# Autodesk Inventor assembly: Chassis_Assembly
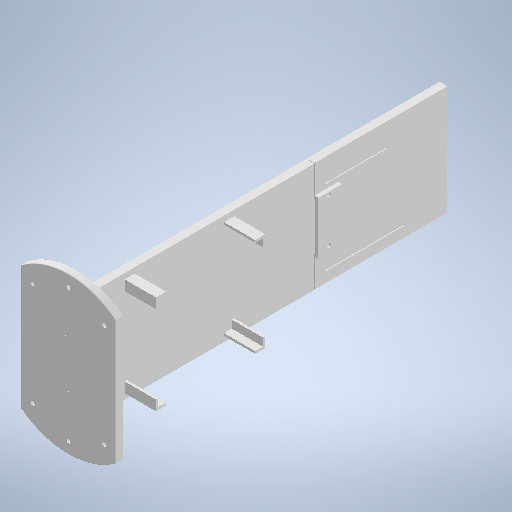
[picture p0: Inventor's stored thumbnail of the model, 512x512]
Saved by Autodesk Inventor 2025 (Build 290162000, 162)
## iProperties
Created: 2024-06-27
Part Number: Chassis_Assembly
Document SubType Name: Assembly
Designer: sml6042
Author: sml6042
## Documents named in this file (4)
- C:\Users\sml6042\Downloads\Chassis_Assembly.iam
- C:\Users\sml6042\Downloads\Chasis_Cap.ipt
- C:\Users\sml6042\Documents\Chasis_Upper_Portion.ipt
- C:\Users\sml6042\Downloads\Chasis_Lower_Portion.ipt
## Components (3 placed, 3 different names)
1. Chasis_Cap:1 — Flush:1, Rigid:1
2. Chasis_Upper_Portion:1 — Flush:1, Rigid:1, Rigid:2
3. Chasis_Lower_Portion:1 — Rigid:2
## Relationships (3: WeldJoint 2, Flush 1)
- Flush:1: Chasis_Cap:1 ↔ Chasis_Upper_Portion:1
- Rigid:1 [WeldJoint]: Chasis_Cap:1 ↔ Chasis_Upper_Portion:1
- Rigid:2 [WeldJoint]: Chasis_Upper_Portion:1 ↔ Chasis_Lower_Portion:1
